# Autodesk Inventor assembly: mucheca
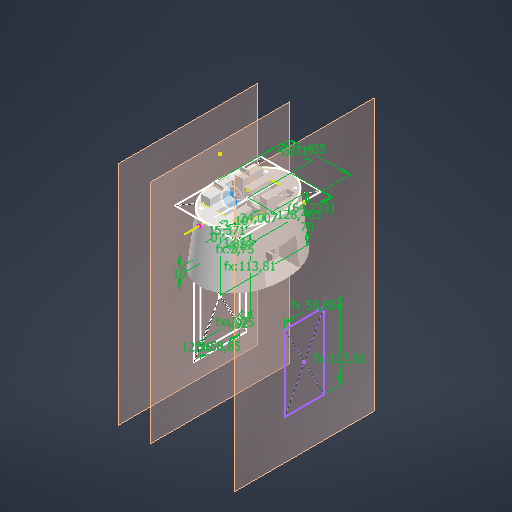
[picture p0: Inventor's stored thumbnail of the model, 512x512]
Saved by Autodesk Inventor 2026.1 (Build 301233020, 233B)
## iProperties
Created: 2026-05-17
Part Number: mucheca
Document SubType Name: Assembly
Designer: user
Author: user
## Documents named in this file (7)
- C:\Users\user\Documents\universidad25-26\TFG\stl\V13\palma\mucheca.iam
- C:\Users\user\Documents\universidad25-26\TFG\mecanismo\v13\antebrazo_v13.ipt
- C:\Users\user\Documents\universidad25-26\TFG\mecanismo\v12\palma\servo_1181_jx.ipt
- C:\Users\user\Documents\universidad25-26\TFG\mecanismo\v12\palma\ruletaServos.ipt
- C:\Users\user\Documents\universidad25-26\TFG\mecanismo\v12\palma\poleaDentro.ipt
- C:\Users\user\Documents\universidad25-26\TFG\mecanismo\v12\palma\poleaFuera.ipt
- C:\Users\user\Documents\universidad25-26\TFG\mecanismo\v13\tapa_antebrazo_v13.ipt
## Components (10 placed, 6 different names)
1. antebrazo_v13:1 — Mate:2, Mate:3, Insert:7, Insert:8, Mate:4, Mate:6, Mate:7, Mate:8
2. servo_1181_jx:2 — Mate:2, Mate:3, Insert:9, Mate:7
3. ruletaServos:2 — Insert:3, Insert:9
4. poleaDentro:2 — Insert:4
5. poleaFuera:2 — Insert:3, Insert:4
6. tapa_antebrazo_v13:1 — Insert:7, Insert:8
7. servo_1181_jx:3 — Mate:4, Mate:6, Mate:8
8. ruletaServos:3
9. poleaDentro:3
10. poleaFuera:3
## Relationships (14: Insert 8, Mate 6)
- Insert:3: ruletaServos:2 ↔ poleaFuera:2
- Insert:4: poleaDentro:2 ↔ poleaFuera:2
- Mate:2: antebrazo_v13:1 ↔ servo_1181_jx:2
- Mate:3: antebrazo_v13:1 ↔ servo_1181_jx:2
- Insert:7: antebrazo_v13:1 ↔ tapa_antebrazo_v13:1
- Insert:8: antebrazo_v13:1 ↔ tapa_antebrazo_v13:1
- Insert:9: servo_1181_jx:2 ↔ ruletaServos:2
- [Insert]: ruletaServos:3 ↔ poleaFuera:3
- [Insert]: poleaDentro:3 ↔ poleaFuera:3
- [Insert]: servo_1181_jx:3 ↔ ruletaServos:3
- Mate:4: antebrazo_v13:1 ↔ servo_1181_jx:3
- Mate:6: antebrazo_v13:1 ↔ servo_1181_jx:3
- Mate:7: antebrazo_v13:1 ↔ servo_1181_jx:2
- Mate:8: antebrazo_v13:1 ↔ servo_1181_jx:3
## Named parameters: d15_d2 = 0 mm, d16_d3 = 0 mm, d17_d14 = 0 mm
